# Autodesk Inventor assembly: flipper_tensioner
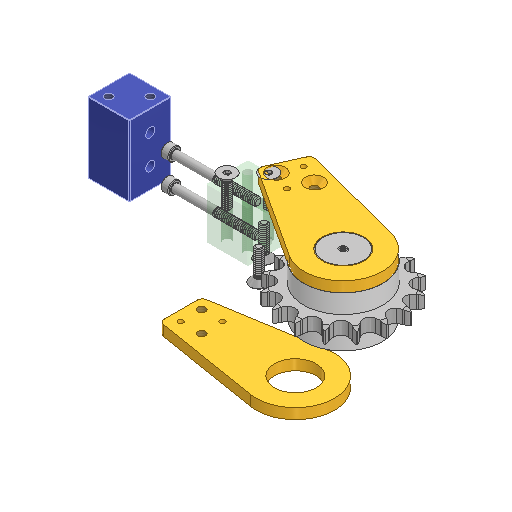
[picture p0: Inventor's stored thumbnail of the model, 512x512]
Saved by Autodesk Inventor 2024 (Build 280153000, 153)
## iProperties
Created: 2023-02-28
Part Number: flipper_tensioner
Document SubType Name: Assembly
Designer: ralph
Author: ralph
## Documents named in this file (9)
- C:\Users\seene\OneDrive\SBRT\Robocup Rescue\Drive\v1\TANK flipper\flipper_tensioner.iam
- C:\Users\seene\OneDrive\SBRT\Robocup Rescue\Drive\v1\TANK flipper\Idler Shaft.ipt
- C:\Users\seene\OneDrive\SBRT\Robocup Rescue\Drive\v1\TANK flipper\Idler Sprocket 16t v12.iam
- C:\Users\seene\OneDrive\SBRT\Robocup Rescue\Drive\v1\TANK flipper\tensioner anchor block.ipt
- C:\Users\seene\OneDrive\SBRT\Robocup Rescue\Drive\v1\TANK flipper\tensioner mobile block.ipt
- C:\Users\seene\OneDrive\SBRT\Robocup Rescue\Drive\v1\TANK flipper\tensioner outside plate.ipt
- C:\Users\seene\OneDrive\SBRT\Robocup Rescue\Drive\v1\TANK flipper\tensioner spacer.ipt
- C:\Users\seene\OneDrive\SBRT\Robocup Rescue\Drive\v1\TANK flipper\91253A245_Black-Oxide Alloy Steel Hex Drive Flat Head Screw v1.ipt
- C:\Users\seene\OneDrive\SBRT\Robocup Rescue\Drive\v1\TANK flipper\90128A229_Zinc-Plated Alloy Steel Socket Head Screw (1) v1.ipt
## Components (13 placed, 8 different names)
1. Idler Shaft:1 — Rotational:3, Mate:1
2. Idler Sprocket 16t v12:1 [sub-assembly] — Rotational:3
3. tensioner anchor block:1 — Rigid:3, Rotational:4, Rigid:9
4. tensioner mobile block:1 — Rigid:2, Rigid:4, Rotational:5
5. tensioner outside plate:1 — Rigid:2, Rigid:7, Rigid:8, Mate:1
6. tensioner spacer:1 — Rigid:3, Rigid:4
7. 91253A245_Black-Oxide Alloy Steel Hex Drive Flat Head Screw v1:2
8. 91253A245_Black-Oxide Alloy Steel Hex Drive Flat Head Screw v1:3
9. 91253A245_Black-Oxide Alloy Steel Hex Drive Flat Head Screw v1:4 — Rigid:7
10. 91253A245_Black-Oxide Alloy Steel Hex Drive Flat Head Screw v1:5 — Rigid:8
11. 90128A229_Zinc-Plated Alloy Steel Socket Head Screw (1) v1:1 — Rotational:4
12. 90128A229_Zinc-Plated Alloy Steel Socket Head Screw (1) v1:2 — Rigid:9
13. tensioner outside plate:2 — Rotational:5
## Relationships (10: WeldJoint 6, RevoluteJoint 3, Mate 1)
- Rigid:2 [WeldJoint]: tensioner mobile block:1 ↔ tensioner outside plate:1
- Rigid:3 [WeldJoint]: tensioner anchor block:1 ↔ tensioner spacer:1
- Rotational:3 [RevoluteJoint]: Idler Shaft:1 ↔ Idler Sprocket 16t v12:1
- Rigid:4 [WeldJoint]: tensioner mobile block:1 ↔ tensioner spacer:1
- Rigid:7 [WeldJoint]: tensioner outside plate:1 ↔ 91253A245_Black-Oxide Alloy Steel Hex Drive Flat Head Screw v1:4
- Rigid:8 [WeldJoint]: tensioner outside plate:1 ↔ 91253A245_Black-Oxide Alloy Steel Hex Drive Flat Head Screw v1:5
- Rotational:4 [RevoluteJoint]: tensioner anchor block:1 ↔ 90128A229_Zinc-Plated Alloy Steel Socket Head Screw (1) v1:1
- Rigid:9 [WeldJoint]: tensioner anchor block:1 ↔ 90128A229_Zinc-Plated Alloy Steel Socket Head Screw (1) v1:2
- Rotational:5 [RevoluteJoint]: tensioner mobile block:1 ↔ tensioner outside plate:2
- Mate:1: Idler Shaft:1 ↔ tensioner outside plate:1
